# Autodesk Inventor assembly: Leg Assembly
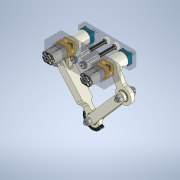
[picture p0: Inventor's stored thumbnail of the model, 180x180]
Saved by Autodesk Inventor 2022 (Build 260153000, 153)
## iProperties
Created: 2021-11-22
Part Number: Leg Assembly
Document SubType Name: Assembly
Designer: JK
Author: JK
## Documents named in this file (15)
- C:\Users\JK\Documents\Inventor\N20 Leg Actuator\CADfiles\Leg Assembly.iam
- C:\Users\JK\Documents\Inventor\N20 Leg Actuator\CADfiles\Brushed DC Motor v8.iam
- C:\Users\JK\Documents\Inventor\N20 Leg Actuator\CADfiles\Base.ipt
- C:\Users\JK\Documents\Inventor\N20 Leg Actuator\CADfiles\LinkA.ipt
- C:\Users\JK\Documents\Inventor\N20 Leg Actuator\CADfiles\Potenciometro10K.iam
- C:\Users\JK\Documents\Inventor\N20 Leg Actuator\CADfiles\PotHolder.ipt
- C:\Users\JK\Documents\Inventor\N20 Leg Actuator\CADfiles\623zz.iam
- C:\Users\JK\Documents\Inventor\N20 Leg Actuator\CADfiles\LinkB.ipt
- C:\Users\JK\Documents\Inventor\N20 Leg Actuator\CADfiles\LinkC.ipt
- C:\Users\JK\Documents\Inventor\N20 Leg Actuator\CADfiles\Rubberfoot.ipt
- C:\Users\JK\Documents\Inventor\N20 Leg Actuator\CADfiles\M3 Locknut.ipt
- C:\Users\JK\Documents\Inventor\N20 Leg Actuator\CADfiles\M3X15.ipt
- C:\Users\JK\Documents\Inventor\N20 Leg Actuator\CADfiles\M3washer.ipt
- C:\Users\JK\Documents\Inventor\N20 Leg Actuator\CADfiles\m3x35.ipt
- C:\Users\JK\Documents\Inventor\N20 Leg Actuator\CADfiles\M3Nut.ipt
## Components (27 placed, 14 different names)
1. Brushed DC Motor v8:1 [sub-assembly] — Coincidencia:2, Coincidencia:3, Ángulo:1, Coincidencia:8
2. Brushed DC Motor v8:2 [sub-assembly] — Coincidencia:4, Ángulo:2, Coincidencia:5, Coincidencia:6, Coincidencia:7, Coincidencia:10
3. Base:1 — Coincidencia:2, Coincidencia:3, Ángulo:1, Coincidencia:4, Ángulo:2, Coincidencia:5, Ángulo:4, Ángulo:5, Coincidencia:14, Coincidencia:36, Ángulo:7, Coincidencia:42
4. LinkA:1 — Coincidencia:6, Coincidencia:7, Nivelación:2, Coincidencia:9, Coincidencia:10, Coincidencia:16, Nivelación:7
5. LinkA:2 — Coincidencia:8, Nivelación:2, Coincidencia:12, Coincidencia:17
6. Potenciometro10K:1 [sub-assembly] — Coincidencia:9, Nivelación:4, Ángulo:3, Ángulo:4, Nivelación:5
7. Potenciometro10K:2 [sub-assembly] — Nivelación:4, Coincidencia:12, Ángulo:3
8. PotHolder:1 — Ángulo:5, Coincidencia:14, Nivelación:5, Coincidencia:36, Coincidencia:37, Coincidencia:38, Coincidencia:39
9. 623zz:1 [sub-assembly] — Coincidencia:16, Nivelación:6, Nivelación:7, Coincidencia:18, Coincidencia:19
10. 623zz:2 [sub-assembly] — Coincidencia:17, Nivelación:6, Coincidencia:21
11. LinkB:1 — Coincidencia:18, Coincidencia:19, Coincidencia:20, Nivelación:8, Coincidencia:22, Coincidencia:24, Coincidencia:26, Coincidencia:30, Coincidencia:35
12. LinkC:1 — Coincidencia:20, Coincidencia:21, Nivelación:8, Nivelación:9, Coincidencia:23, Coincidencia:25, Nivelación:19, Coincidencia:43
13. 623zz:3 [sub-assembly] — Coincidencia:22, Nivelación:9
14. Rubberfoot:1 — Coincidencia:23, Nivelación:19, Coincidencia:43
15. Unbrako Hex Socket Cap - Metric M3 x 25:1 — Coincidencia:24, Nivelación:11, Coincidencia:27, Coincidencia:32
16. Unbrako Hex Socket Cap - Metric M3 x 25:2 — Coincidencia:25, Nivelación:12, Coincidencia:28, Coincidencia:31
17. Unbrako Hex Socket Cap - Metric M3 x 25:3 — Coincidencia:26, Nivelación:11, Nivelación:12, Coincidencia:29, Coincidencia:33, Coincidencia:34
18. M3 Locknut:1 — Coincidencia:28, Nivelación:13
19. M3 Locknut:2 — Coincidencia:27, Nivelación:13, Nivelación:14
20. M3 Locknut:3 — Coincidencia:29, Nivelación:14, Coincidencia:30
21. M3washer:1 — Coincidencia:33, Coincidencia:34, Nivelación:15
22. M3washer:2 — Coincidencia:32, Nivelación:16, Coincidencia:35
23. M3washer:3 — Coincidencia:31, Nivelación:15, Nivelación:16
24. m3x35:1 — Coincidencia:37, Nivelación:17, Coincidencia:39, Coincidencia:40
25. m3x35:2 — Coincidencia:38, Nivelación:17, Coincidencia:41
26. M3Nut:1 — Coincidencia:40, Ángulo:6, Ángulo:7, Nivelación:18, Coincidencia:42
27. M3Nut:2 — Coincidencia:41, Ángulo:6, Nivelación:18
## Relationships (62: Mate 39, Flush 16, Angle 7)
- Coincidencia:2 [Mate]: Brushed DC Motor v8:1 ↔ Base:1
- Coincidencia:3 [Mate]: Brushed DC Motor v8:1 ↔ Base:1
- Ángulo:1 [Angle] (0 deg): Brushed DC Motor v8:1 ↔ Base:1
- Coincidencia:4 [Mate]: Brushed DC Motor v8:2 ↔ Base:1
- Ángulo:2 [Angle] (0 deg): Brushed DC Motor v8:2 ↔ Base:1
- Coincidencia:5 [Mate]: Brushed DC Motor v8:2 ↔ Base:1
- Coincidencia:6 [Mate]: Brushed DC Motor v8:2 ↔ LinkA:1
- Coincidencia:7 [Mate]: Brushed DC Motor v8:2 ↔ LinkA:1
- Coincidencia:8 [Mate]: Brushed DC Motor v8:1 ↔ LinkA:2
- Nivelación:2 [Flush]: LinkA:1 ↔ LinkA:2
- Coincidencia:9 [Mate]: LinkA:1 ↔ Potenciometro10K:1
- Coincidencia:10 [Mate]: Brushed DC Motor v8:2 ↔ LinkA:1
- Nivelación:4 [Flush]: Potenciometro10K:1 ↔ Potenciometro10K:2
- Coincidencia:12 [Mate]: LinkA:2 ↔ Potenciometro10K:2
- Ángulo:3 [Angle] (0 deg): Potenciometro10K:1 ↔ Potenciometro10K:2
- Ángulo:4 [Angle] (0 deg): Base:1 ↔ Potenciometro10K:1
- Ángulo:5 [Angle] (0 deg): Base:1 ↔ PotHolder:1
- Coincidencia:14 [Mate]: Base:1 ↔ PotHolder:1
- Nivelación:5 [Flush]: Potenciometro10K:1 ↔ PotHolder:1
- Coincidencia:16 [Mate]: LinkA:1 ↔ 623zz:1
- Coincidencia:17 [Mate]: LinkA:2 ↔ 623zz:2
- Nivelación:6 [Flush]: 623zz:1 ↔ 623zz:2
- Nivelación:7 [Flush]: LinkA:1 ↔ 623zz:1
- Coincidencia:18 [Mate]: 623zz:1 ↔ LinkB:1
- Coincidencia:19 [Mate] (0.15 mm): 623zz:1 ↔ LinkB:1
- Coincidencia:20 [Mate]: LinkB:1 ↔ LinkC:1
- Coincidencia:21 [Mate]: 623zz:2 ↔ LinkC:1
- Nivelación:8 [Flush]: LinkB:1 ↔ LinkC:1
- Coincidencia:22 [Mate]: LinkB:1 ↔ 623zz:3
- Nivelación:9 [Flush]: LinkC:1 ↔ 623zz:3
- Coincidencia:23 [Mate]: LinkC:1 ↔ Rubberfoot:1
- Coincidencia:24 [Mate]: LinkB:1 ↔ Unbrako Hex Socket Cap - Metric M3 x 25:1
- Coincidencia:25 [Mate]: LinkC:1 ↔ Unbrako Hex Socket Cap - Metric M3 x 25:2
- Coincidencia:26 [Mate]: LinkB:1 ↔ Unbrako Hex Socket Cap - Metric M3 x 25:3
- Nivelación:11 [Flush]: Unbrako Hex Socket Cap - Metric M3 x 25:1 ↔ Unbrako Hex Socket Cap - Metric M3 x 25:3
- Nivelación:12 [Flush]: Unbrako Hex Socket Cap - Metric M3 x 25:2 ↔ Unbrako Hex Socket Cap - Metric M3 x 25:3
- Coincidencia:27 [Mate]: Unbrako Hex Socket Cap - Metric M3 x 25:1 ↔ M3 Locknut:2
- Coincidencia:28 [Mate]: Unbrako Hex Socket Cap - Metric M3 x 25:2 ↔ M3 Locknut:1
- Coincidencia:29 [Mate]: Unbrako Hex Socket Cap - Metric M3 x 25:3 ↔ M3 Locknut:3
- Nivelación:13 [Flush]: M3 Locknut:1 ↔ M3 Locknut:2
- Nivelación:14 [Flush]: M3 Locknut:2 ↔ M3 Locknut:3
- Coincidencia:30 [Mate]: LinkB:1 ↔ M3 Locknut:3
- Coincidencia:31 [Mate]: Unbrako Hex Socket Cap - Metric M3 x 25:2 ↔ M3washer:3
- Coincidencia:32 [Mate]: Unbrako Hex Socket Cap - Metric M3 x 25:1 ↔ M3washer:2
- Coincidencia:33 [Mate]: Unbrako Hex Socket Cap - Metric M3 x 25:3 ↔ M3washer:1
- Coincidencia:34 [Mate]: Unbrako Hex Socket Cap - Metric M3 x 25:3 ↔ M3washer:1
- Nivelación:15 [Flush]: M3washer:1 ↔ M3washer:3
- Nivelación:16 [Flush]: M3washer:2 ↔ M3washer:3
- Coincidencia:35 [Mate]: LinkB:1 ↔ M3washer:2
- Coincidencia:36 [Mate]: Base:1 ↔ PotHolder:1
- Coincidencia:37 [Mate]: PotHolder:1 ↔ m3x35:1
- Coincidencia:38 [Mate]: PotHolder:1 ↔ m3x35:2
- Nivelación:17 [Flush]: m3x35:1 ↔ m3x35:2
- Coincidencia:39 [Mate]: PotHolder:1 ↔ m3x35:1
- Coincidencia:40 [Mate]: m3x35:1 ↔ M3Nut:1
- Coincidencia:41 [Mate]: m3x35:2 ↔ M3Nut:2
- Ángulo:6 [Angle] (0 deg): M3Nut:1 ↔ M3Nut:2
- Ángulo:7 [Angle] (0 deg): Base:1 ↔ M3Nut:1
- Nivelación:18 [Flush]: M3Nut:1 ↔ M3Nut:2
- Coincidencia:42 [Mate]: Base:1 ↔ M3Nut:1
- Nivelación:19 [Flush]: LinkC:1 ↔ Rubberfoot:1
- Coincidencia:43 [Mate]: LinkC:1 ↔ Rubberfoot:1
